# Autodesk Inventor assembly: Complete_Assembly
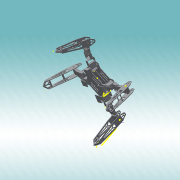
[picture p0: Inventor's stored thumbnail of the model, 180x180]
Saved by Autodesk Inventor 2019 (Build 230136000, 136)
## iProperties
Created: 2019-02-11
Part Number: Complete_Assembly
Document SubType Name: Assembly
Designer: USUARIO
Author: USUARIO
## Documents named in this file (6)
- D:\Users\Documents\Inventor parts\Structure_Charlotte\Structure_Charlotte\Complete_Assembly.iam
- D:\Users\Documents\Inventor parts\Structure_Charlotte\Structure_Charlotte\Complete_leg_assembly.iam
- D:\Users\Documents\Inventor parts\Structure_Charlotte\Structure_Charlotte\Superior_Base.ipt
- D:\Users\Documents\Inventor parts\Structure_Charlotte\Structure_Charlotte\lipo_1.ipt
- D:\Users\Documents\Inventor parts\Structure_Charlotte\Structure_Charlotte\center_joint.ipt
- D:\Users\Documents\Inventor parts\Structure_Charlotte\Structure_Charlotte\Middle_base.ipt
## Components (15 placed, 5 different names)
1. Complete_leg_assembly:1 [sub-assembly] — Rigid:13, Rigid:14, Rigid:15
2. Superior_Base:1 — Rigid:10, Rigid:11, Rigid:12, Rigid:13
3. Complete_leg_assembly:2 [sub-assembly] — Rigid:11, Rigid:17
4. Superior_Base:2 — Rigid:6, Rigid:7, Rigid:8, Rigid:9, Rigid:14
5. Complete_leg_assembly:3 [sub-assembly] — Rigid:12, Rigid:16
6. Complete_leg_assembly:4 [sub-assembly] — Rigid:10, Rigid:18
7. lipo_1:1 — Rigid:9
8. lipo_1:2 — Rigid:8
9. lipo_1:3 — Rigid:7
10. lipo_1:4 — Rigid:6
11. center_joint:1 — Rigid:17
12. center_joint:2 — Rigid:18
13. center_joint:3 — Rigid:16, Rigid:19
14. center_joint:4 — Rigid:15
15. Middle_base:1 — Rigid:19
## Relationships (14: WeldJoint 14)
- Rigid:6 [WeldJoint]: Superior_Base:2 ↔ lipo_1:4
- Rigid:7 [WeldJoint]: Superior_Base:2 ↔ lipo_1:3
- Rigid:8 [WeldJoint]: Superior_Base:2 ↔ lipo_1:2
- Rigid:9 [WeldJoint]: Superior_Base:2 ↔ lipo_1:1
- Rigid:10 [WeldJoint]: Superior_Base:1 ↔ Complete_leg_assembly:4
- Rigid:11 [WeldJoint]: Superior_Base:1 ↔ Complete_leg_assembly:2
- Rigid:12 [WeldJoint]: Superior_Base:1 ↔ Complete_leg_assembly:3
- Rigid:13 [WeldJoint]: Complete_leg_assembly:1 ↔ Superior_Base:1
- Rigid:14 [WeldJoint]: Complete_leg_assembly:1 ↔ Superior_Base:2
- Rigid:15 [WeldJoint]: Complete_leg_assembly:1 ↔ center_joint:4
- Rigid:16 [WeldJoint]: Complete_leg_assembly:3 ↔ center_joint:3
- Rigid:17 [WeldJoint]: Complete_leg_assembly:2 ↔ center_joint:1
- Rigid:18 [WeldJoint]: Complete_leg_assembly:4 ↔ center_joint:2
- Rigid:19 [WeldJoint]: center_joint:3 ↔ Middle_base:1
